# Autodesk Inventor assembly: Baugruppe2
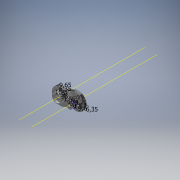
[picture p0: Inventor's stored thumbnail of the model, 180x180]
Saved by Autodesk Inventor 2018.3 (Build 223284000, 284)
## iProperties
Created: 2018-07-27
Part Number: Baugruppe2
Material: Generisch
Document SubType Name: Assembly
Designer: JochenAlt
Author: JochenAlt
## Documents named in this file (3)
- D:\Projects\FlowerPot\CAD\Beltdrive\BeltDriveConstruction.iam
- D:\Projects\FlowerPot\CAD\Beltdrive\Konstruktions-Assistent\Übertragung des Zahnriemens1.iam
- D:\Projects\FlowerPot\CAD\Beltdrive\BeltDriveConstruction\Konstruktions-Assistent\Übertragung des Zahnriemens1.iam
## Components (2 placed, 1 different names)
1. Übertragung des Zahnriemens:3 [sub-assembly] — Passend:8, Passend:9, Passend:10, Passend:11, Drehung:1
2. Übertragung des Zahnriemens:4 [sub-assembly] — Passend:9, Passend:11, Drehung:1
## Relationships (5: Mate 4, RelateRotation 1)
- Passend:8 [Mate]: Übertragung des Zahnriemens:3
- Passend:9 [Mate]: Übertragung des Zahnriemens:3 ↔ Übertragung des Zahnriemens:4
- Passend:10 [Mate]: Übertragung des Zahnriemens:3
- Passend:11 [Mate]: Übertragung des Zahnriemens:3 ↔ Übertragung des Zahnriemens:4
- Drehung:1 [RelateRotation] (-1 ul): Übertragung des Zahnriemens:3 ↔ Übertragung des Zahnriemens:4
